# Autodesk Inventor assembly: KBRI-16
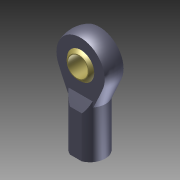
[picture p0: Inventor's stored thumbnail of the model, 180x180]
Saved by Autodesk Inventor 2011 (Build 150239000, 239)
## iProperties
Category: Plastic Bearings
Created: 2007-11-11
Part Number: KBRI-16
Catalog Web Link: http://www.igus.com/igcat/ig_cat1.asp?p=ig_24_2.gif
Description: igubal Rod End Bearing
Vendor: igus
Document SubType Name: Assembly
Mass: 185.736 g
Surface Area: 350.339 cm^2
Volume: 160.703 cm^3
Density: 1.15577 g/cm^3
Project: FIRST
Title: igubal Rod End Bearing
Author: Autodesk, Inc.
## Documents named in this file (3)
- R:\2012\Inventor\vkop\Plastic-Bearings\Plastic Bearings_igus_KBRI-16.iam
- R:\2012\Inventor\vkop\Plastic-Bearings\KBRI-16_Housing.ipt
- R:\2012\Inventor\vkop\Plastic-Bearings\KBRI-16_Spherical bearing.ipt
## Components (2 placed, 2 different names)
1. KBRI-16_Housing:1 — Mate:1, Angle:1
2. KBRI-16_Spherical bearing:1 — Mate:1, Angle:1
## Relationships (2: Mate 1, Angle 1)
- Mate:1: KBRI-16_Housing:1 ↔ KBRI-16_Spherical bearing:1
- Angle:1 (0 deg): KBRI-16_Housing:1 ↔ KBRI-16_Spherical bearing:1
